# Autodesk Inventor assembly: electronics
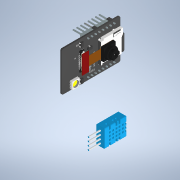
[picture p0: Inventor's stored thumbnail of the model, 180x180]
Saved by Autodesk Inventor 2022 (Build 260153000, 153)
## iProperties
Created: 2022-08-08
Part Number: electronics
Document SubType Name: Assembly
Designer: thoma
Author: thoma
## Documents named in this file (3)
- C:\Users\thoma\OneDrive\Documents\CREATION\Serre\electronics.iam
- C:\Users\thoma\OneDrive\Documents\CREATION\Serre\ESP3-CAM.ipt
- C:\Users\thoma\OneDrive\Documents\CREATION\Serre\dht11.ipt
## Components (2 placed, 2 different names)
1. ESP3-CAM:1 — Mate:1, Flush:1, Flush:2
2. dht11:1 — Mate:1, Flush:1, Flush:2
## Relationships (3: Flush 2, Mate 1)
- Mate:1 (30 mm): ESP3-CAM:1 ↔ dht11:1
- Flush:1: ESP3-CAM:1 ↔ dht11:1
- Flush:2: ESP3-CAM:1 ↔ dht11:1
